# Autodesk Inventor assembly: Reloj Digital
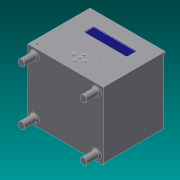
[picture p0: Inventor's stored thumbnail of the model, 180x180]
Saved by Autodesk Inventor 2019 (Build 230136000, 136)
## iProperties
Created: 2023-11-26
Part Number: Reloj Digital
Document SubType Name: Assembly
Designer: Familia CS
Author: Familia CS
## Documents named in this file (5)
- C:\Users\Familia CS\Mi unidad (hermesjcc34@gmail.com)\Mis Proyectos\Reloj Digital LCD 16 x 4\Inventor\PCB\Reloj digital\Reloj Digital.iam
- C:\Users\Familia CS\Mi unidad (hermesjcc34@gmail.com)\Mis Proyectos\Reloj Digital LCD 16 x 4\Inventor\PCB\Front\Tapa Front editado.ipt
- C:\Users\Familia CS\Mi unidad (hermesjcc34@gmail.com)\Mis Proyectos\Reloj Digital LCD 16 x 4\Inventor\PCB\Front\PCB\PCB Front.ipt
- C:\Users\Familia CS\Mi unidad (hermesjcc34@gmail.com)\Mis Proyectos\Reloj Digital LCD 16 x 4\Inventor\Pulsadores\3D\Tools Pulsadores editado.ipt
- C:\Users\Familia CS\Mi unidad (hermesjcc34@gmail.com)\Mis Proyectos\Reloj Digital LCD 16 x 4\Altium\Reloj Digital Down\PCB\PCB Down.iam
## Components (4 placed, 4 different names)
1. Tapa Front editado:1 — Rotational:2, Rotational:4
2. PCB Front:1 — Rotational:2, Rotational:3
3. Tools Pulsadores editado:1 — Rotational:3
4. PCB Down:1 [sub-assembly] — Rotational:4
## Relationships (3: RevoluteJoint 3)
- Rotational:2 [RevoluteJoint]: Tapa Front editado:1 ↔ PCB Front:1
- Rotational:3 [RevoluteJoint]: PCB Front:1 ↔ Tools Pulsadores editado:1
- Rotational:4 [RevoluteJoint]: Tapa Front editado:1 ↔ PCB Down:1
